# Autodesk Inventor assembly: Design5
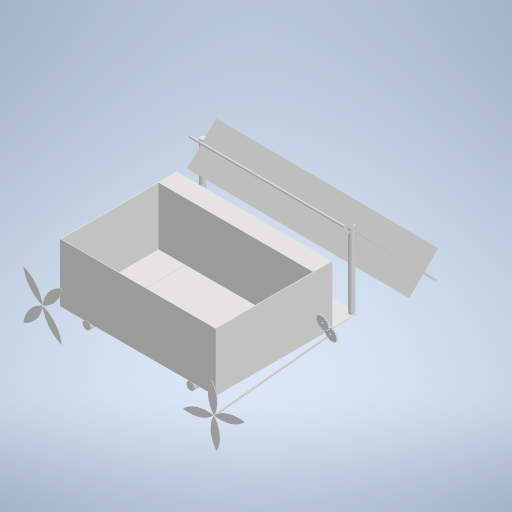
[picture p0: Inventor's stored thumbnail of the model, 512x512]
Saved by Autodesk Inventor 2024 (Build 280153000, 153)
## iProperties
Created: 2024-09-18
Part Number: Design5
Document SubType Name: Assembly
Designer: srira
Author: srira
## Documents named in this file (6)
- C:\Users\srira\Documents\IITGN\3rd year\Sem5\ES408\Tentative Model\Design5.iam
- C:\Users\srira\Documents\IITGN\3rd year\Sem5\ES408\Tentative Model\PVC.ipt
- C:\Users\srira\Documents\IITGN\3rd year\Sem5\ES408\Tentative Model\Distanced Top Bin.ipt
- C:\Users\srira\Documents\IITGN\3rd year\Sem5\ES408\Tentative Model\Layered Belt.ipt
- C:\Users\srira\Documents\IITGN\3rd year\Sem5\ES408\Tentative Model\ranpro.ipt
- C:\Users\srira\Documents\IITGN\3rd year\Sem5\ES408\Tentative Model\Ger.ipt
## Components (10 placed, 5 different names)
1. PVC:1
2. PVC:2
3. Distanced Top Bin:1
4. Layered Belt:1
5. ranpro:1 — Mate:4
6. ranpro:2 — Mate:2
7. Ger:1 — Mate:1, Mate:2
8. Ger:2 — Mate:1
9. Ger:3 — Mate:3
10. Ger:4 — Mate:3, Mate:4
## Relationships (4: Mate 4)
- Mate:1: Ger:1 ↔ Ger:2
- Mate:2: ranpro:2 ↔ Ger:1
- Mate:3: Ger:3 ↔ Ger:4
- Mate:4: ranpro:1 ↔ Ger:4
